# Autodesk Inventor assembly: Servo_Bracket
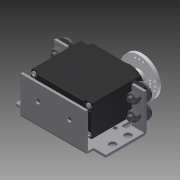
[picture p0: Inventor's stored thumbnail of the model, 180x180]
Saved by Autodesk Inventor 2015 (Build 190159000, 159)
## iProperties
Created: 2015-05-21
Part Number: Servo_Bracket
Document SubType Name: Assembly
Designer: Quinn
Author: Quinn
## Documents named in this file (6)
- C:\Users\Quinn\Desktop\3DCNC Design\InventorModels\Servo_Bracket.iam
- C:\Users\Quinn\Desktop\3DCNC Design\InventorModels\Metal\Brackets\asb-04-ServoMount.ipt
- C:\Users\Quinn\Desktop\3DCNC Design\InventorModels\Electronics\Servo\standard_servo.iam
- C:\Users\Quinn\Desktop\3DCNC Design\InventorModels\Hardware\Washers\Washer Flat 3mm.ipt
- C:\Users\Quinn\Desktop\3DCNC Design\InventorModels\Hardware\Screws\M3 X 8 LG PHMS (PHS-00).ipt
- C:\Users\Quinn\Desktop\3DCNC Design\InventorModels\Hardware\Nuts\Nut Hex M3.ipt
## Components (14 placed, 5 different names)
1. asb-04-ServoMount:1 — Insert:1, Insert:10, Insert:11, Mate:1, Mate:2
2. standard_servo:1 [sub-assembly] — Insert:1, Insert:2, Insert:3, Insert:4, Insert:5
3. Washer Flat 3mm:1 — Insert:3, Insert:7
4. Washer Flat 3mm:2 — Insert:4, Insert:9
5. Washer Flat 3mm:3 — Insert:2, Insert:6
6. Washer Flat 3mm:4 — Insert:5, Insert:8
7. M3 X 8 LG PHMS (PHS-00):1 — Insert:8
8. M3 X 8 LG PHMS (PHS-00):2 — Insert:7
9. M3 X 8 LG PHMS (PHS-00):3 — Insert:6
10. M3 X 8 LG PHMS (PHS-00):4 — Insert:9
11. Nut Hex M3:1 — Insert:10
12. Nut Hex M3:2 — Insert:11
13. Nut Hex M3:3 — Mate:1
14. Nut Hex M3:4 — Mate:2
## Relationships (13: Insert 11, Mate 2)
- Insert:1: asb-04-ServoMount:1 ↔ standard_servo:1
- Insert:2: standard_servo:1 ↔ Washer Flat 3mm:3
- Insert:3: standard_servo:1 ↔ Washer Flat 3mm:1
- Insert:4: standard_servo:1 ↔ Washer Flat 3mm:2
- Insert:5: standard_servo:1 ↔ Washer Flat 3mm:4
- Insert:6: Washer Flat 3mm:3 ↔ M3 X 8 LG PHMS (PHS-00):3
- Insert:7: Washer Flat 3mm:1 ↔ M3 X 8 LG PHMS (PHS-00):2
- Insert:8: Washer Flat 3mm:4 ↔ M3 X 8 LG PHMS (PHS-00):1
- Insert:9: Washer Flat 3mm:2 ↔ M3 X 8 LG PHMS (PHS-00):4
- Insert:10: asb-04-ServoMount:1 ↔ Nut Hex M3:1
- Insert:11: asb-04-ServoMount:1 ↔ Nut Hex M3:2
- Mate:1 (1.016 mm): asb-04-ServoMount:1 ↔ Nut Hex M3:3
- Mate:2 (1.016 mm): asb-04-ServoMount:1 ↔ Nut Hex M3:4
